# Autodesk Inventor assembly: Chuck with BBM Staging Plate
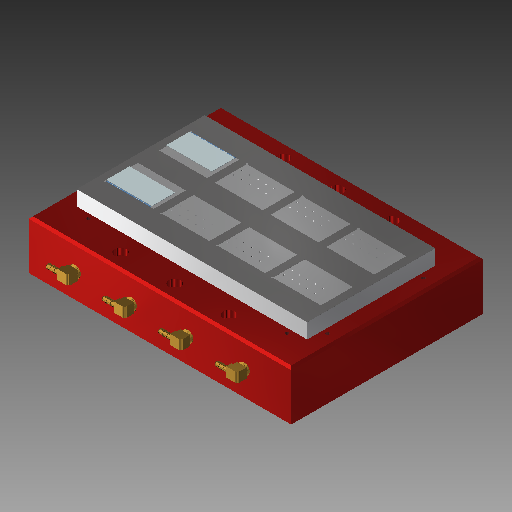
[picture p0: Inventor's stored thumbnail of the model, 512x512]
Saved by Autodesk Inventor 2019.4 (Build 234330000, 330)
## iProperties
Created: 2021-02-26
Part Number: Chuck with BBM Staging Plate
Document SubType Name: Assembly
Designer: caleb
Author: caleb
## Documents named in this file (3)
- C:\Users\cfang\Desktop\nebraska-silicon-lab\Hardware\ETL\Module Assembly\Chuck with BBM Staging Plate.iam
- C:\Users\cfang\Desktop\nebraska-silicon-lab\Hardware\ETL\Module Assembly\Chuck - Multipocket\Chuck Assembly.iam
- C:\Users\cfang\Desktop\nebraska-silicon-lab\Hardware\ETL\Module Assembly\BBM Staging Plate\BBM Staging Plate Assembly.iam
## Components (2 placed, 2 different names)
1. Chuck Assembly:1 [sub-assembly] — Mate:1, Angle:1, Tangent:1, Tangent:2
2. BBM Staging Plate Assembly:1 [sub-assembly] — Mate:1, Angle:1, Tangent:1, Tangent:2
## Relationships (4: Tangent 2, Mate 1, Angle 1)
- Mate:1: Chuck Assembly:1 ↔ BBM Staging Plate Assembly:1
- Angle:1 (0 deg): Chuck Assembly:1 ↔ BBM Staging Plate Assembly:1
- Tangent:1: Chuck Assembly:1 ↔ BBM Staging Plate Assembly:1
- Tangent:2: Chuck Assembly:1 ↔ BBM Staging Plate Assembly:1
